# Autodesk Inventor assembly: Ortur Laser Master 2 Pro S2 LF
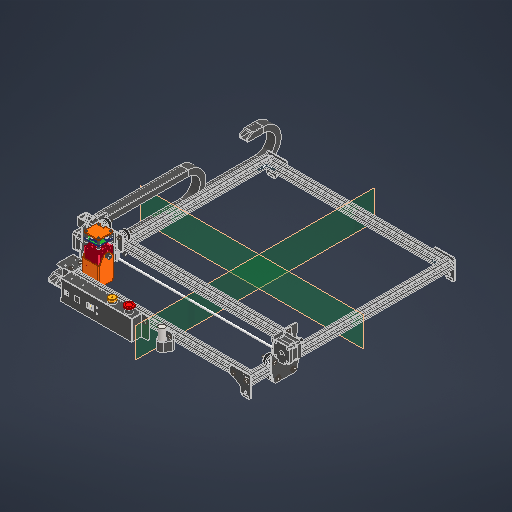
[picture p0: Inventor's stored thumbnail of the model, 512x512]
Saved by Autodesk Inventor 2025 (Build 290162000, 162)
## iProperties
Created: 2024-11-17
Part Number: Ortur Laser Master 2 Pro S2 LF
Description: STEP AP214
Document SubType Name: Assembly
Designer: Admin
Title: ortur_laser_no_fan.stp
Author: Admin
Revision Number: ANY
Sending System: Autodesk Inventor 2025
Preprocessor: ST-DEVELOPER v20
## Documents named in this file (10)
- V:\INVENTOR\laser\ortur\ortur_laser_master_s2_information\3D model\ortur_s2\ortur_s2.iam
- V:\INVENTOR\laser\ortur\ortur_laser_master_s2_information\3D model\ortur_s2\Base.iam
- V:\INVENTOR\laser\ortur\ortur_laser_master_s2_information\3D model\ortur_s2\Chariot Y.iam
- V:\INVENTOR\laser\ortur\ortur_laser_master_s2_information\3D model\ortur_s2\Chariot X.iam
- V:\INVENTOR\laser\ortur\ortur_laser_master_s2_information\3D model\ortur_s2\Module Laser LU2-4-LF_Stock.iam
- V:\INVENTOR\laser\ortur\ortur_laser_master_s2_information\3D model\ortur_s2\Chaine porte cable 1_260.ipt
- V:\INVENTOR\laser\ortur\ortur_laser_master_s2_information\3D model\ortur_s2\Chaine porte cable 2.ipt
- V:\INVENTOR\laser\ortur\ortur_laser_master_s2_information\3D model\ortur_s2\Chaine porte cable 1_xxx.ipt
- V:\INVENTOR\laser\ortur\ortur_laser_master_s2_information\3D model\ortur_s2\Chaine porte cable 1_xxx2.ipt
- V:\INVENTOR\laser\ortur\ortur_laser_master_s2_information\inventor\Ortur Laser Master 2 Pro S2 LF\peg_board.ipt
## Components (10 placed, 10 different names)
1. Base_1 [sub-assembly] — Flush:1
2. Chariot Y_2 [sub-assembly]
3. Chariot X_3 [sub-assembly]
4. Module Laser LU2-4-LF_Stock_4 [sub-assembly]
5. Chaine porte cable 1_260_5
6. Chaine porte cable 2_6
7. Chaine porte cable 2_7
8. Chaine porte cable 1_xxx_8
9. Chaine porte cable 1_xxx2_9
10. peg_board:1 — Flush:1
## Relationships (1: Flush 1)
- Flush:1: Base_1 ↔ peg_board:1
